# Autodesk Inventor assembly: Assembly21
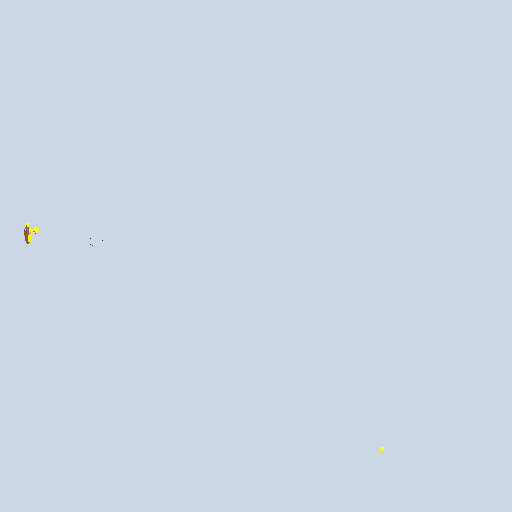
[picture p0: Inventor's stored thumbnail of the model, 512x512]
Saved by Autodesk Inventor 2024.1 (Build 281209000, 209)
## iProperties
Created: 2023-11-10
Part Number: Assembly21
Document SubType Name: Assembly
Designer: luvag
Author: luvag
## Documents named in this file (3)
- C:\Users\luvag\Desktop\Assembly21.iam
- C:\Users\luvag\Desktop\Assembly20.iam
- C:\Users\luvag\Desktop\final_boat.ipt
## Components (2 placed, 2 different names)
1. Assembly20:1 [sub-assembly]
2. final_boat:1
## Relationships (1: Mate 1)
- [Mate]: Assembly20:1 ↔ final_boat:1
